# Autodesk Inventor assembly: WaagePlexi
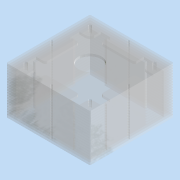
[picture p0: Inventor's stored thumbnail of the model, 180x180]
Saved by Autodesk Inventor 2022 (Build 260153000, 153)
## iProperties
Created: 2021-12-03
Part Number: WaagePlexi
Document SubType Name: Assembly
Designer: domin
Author: domin
## Documents named in this file (5)
- D:\Sync\Hivemind\1-MCI-Unterlagen\Master\Semester 3\Projekt 2\011_Kartesischer_Roboter_Modul\07-CAD Files\04-Waage\WaagePlexi.iam
- D:\Sync\Hivemind\1-MCI-Unterlagen\Master\Semester 3\Projekt 2\011_Kartesischer_Roboter_Modul\07-CAD Files\04-Waage\WaagePlexiOben1.ipt
- D:\Sync\Hivemind\1-MCI-Unterlagen\Master\Semester 3\Projekt 2\011_Kartesischer_Roboter_Modul\07-CAD Files\04-Waage\WaagePlexiOben2.ipt
- D:\Sync\Hivemind\1-MCI-Unterlagen\Master\Semester 3\Projekt 2\011_Kartesischer_Roboter_Modul\07-CAD Files\04-Waage\WaagePlexiOben3.ipt
- D:\Sync\Hivemind\1-MCI-Unterlagen\Master\Semester 3\Projekt 2\011_Kartesischer_Roboter_Modul\07-CAD Files\04-Waage\WaagePlexiMittelsteuck.ipt
## Components (20 placed, 4 different names)
1. WaagePlexiOben1:1 — Flush:1, Flush:2, Flush:3, Flush:4, Flush:5, Mate:1, Flush:6, Flush:7, Flush:8, Flush:9, Mate:3
2. WaagePlexiOben2:1 — Flush:4, Flush:5, Mate:1, Mate:2
3. WaagePlexiOben3:1 — Flush:6, Flush:7, Mate:2
4. WaagePlexiMittelsteuck:1 — Flush:8, Flush:9, Mate:3
5. WaagePlexiMittelsteuck:2
6. WaagePlexiMittelsteuck:3
7. WaagePlexiMittelsteuck:4
8. WaagePlexiMittelsteuck:5
9. WaagePlexiMittelsteuck:6
10. WaagePlexiMittelsteuck:7
11. WaagePlexiMittelsteuck:8
12. WaagePlexiMittelsteuck:9
13. WaagePlexiMittelsteuck:10
14. WaagePlexiMittelsteuck:11
15. WaagePlexiMittelsteuck:12
16. WaagePlexiMittelsteuck:13
17. WaagePlexiMittelsteuck:14
18. WaagePlexiMittelsteuck:15
19. WaagePlexiMittelsteuck:16
20. WaagePlexiMittelsteuck:17
## Component patterns: (17 elements, first: WaagePlexiMittelsteuck:1)
## Relationships (12: Flush 9, Mate 3)
- Flush:1: WaagePlexiOben1:1
- Flush:2: WaagePlexiOben1:1
- Flush:3: WaagePlexiOben1:1
- Flush:4: WaagePlexiOben1:1 ↔ WaagePlexiOben2:1
- Flush:5: WaagePlexiOben1:1 ↔ WaagePlexiOben2:1
- Mate:1: WaagePlexiOben1:1 ↔ WaagePlexiOben2:1
- Flush:6: WaagePlexiOben1:1 ↔ WaagePlexiOben3:1
- Flush:7: WaagePlexiOben1:1 ↔ WaagePlexiOben3:1
- Mate:2: WaagePlexiOben2:1 ↔ WaagePlexiOben3:1
- Flush:8: WaagePlexiOben1:1 ↔ WaagePlexiMittelsteuck:1
- Flush:9: WaagePlexiOben1:1 ↔ WaagePlexiMittelsteuck:1
- Mate:3: WaagePlexiOben1:1 ↔ WaagePlexiMittelsteuck:1
